# Autodesk Inventor assembly: B_Legs0
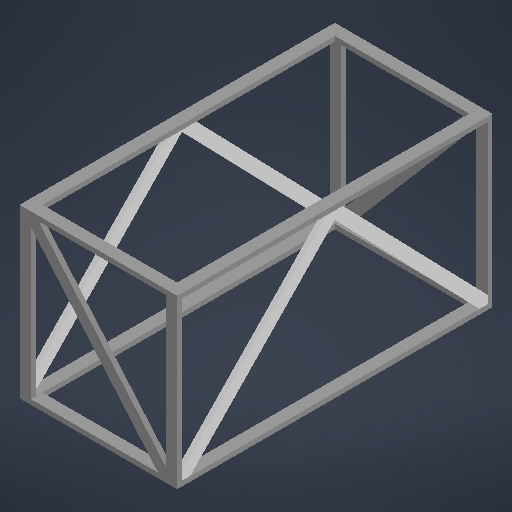
[picture p0: Inventor's stored thumbnail of the model, 512x512]
Saved by Autodesk Inventor 2026 (Build 300175000, 175)
## iProperties
Created: 2024-09-19
Part Number: B_Legs0
Document SubType Name: Assembly
Designer: User
Author: User
## Documents named in this file (7)
- C:\Users\trott\Documents\UofSC-ASME-Tiger-Burn-Design-2025\CAD\Legs\Back Foot\B_Feet.iam
- C:\Users\trott\Documents\UofSC-ASME-Tiger-Burn-Design-2025\CAD\Legs\Back Foot\2x4x120.ipt
- C:\Users\trott\Documents\UofSC-ASME-Tiger-Burn-Design-2025\CAD\Legs\Back Foot\2x4x42.ipt
- C:\Users\trott\Documents\UofSC-ASME-Tiger-Burn-Design-2025\CAD\Legs\Back Foot\2x4x48.ipt
- C:\Users\trott\Documents\UofSC-ASME-Tiger-Burn-Design-2025\CAD\Legs\Back Foot\S_2x4x44.ipt
- C:\Users\trott\Documents\UofSC-ASME-Tiger-Burn-Design-2025\CAD\Legs\Back Foot\S_2x4x65.081.ipt
- C:\Users\trott\Documents\UofSC-ASME-Tiger-Burn-Design-2025\CAD\Legs\Back Foot\S_2x4x68.525.ipt
## Components (18 placed, 6 different names)
1. 2x4x120:1 — Flush:1, Flush:2, Flush:3, Flush:4, Flush:5, Flush:8, Mate:3, Flush:10, Flush:12, Flush:13, Flush:14
2. 2x4x120:2 — Mate:1, Flush:1, Flush:2, Flush:3, Mate:2, Flush:6, Flush:7, Mate:5, Flush:9, Flush:11, Flush:15, Flush:16
3. 2x4x42:1 — Flush:4, Flush:5
4. 2x4x42:2 — Mate:2, Flush:6, Flush:7, Mate:4
5. 2x4x48:1 — Flush:8, Flush:13, Flush:14, Mate:7, Flush:17, Flush:20, Mate:15
6. 2x4x48:2 — Mate:5, Flush:15, Flush:16, Mate:6, Flush:18, Flush:19, Flush:27, Mate:20
7. 2x4x48:3 — Mate:4, Flush:9, Flush:11, Mate:19
8. 2x4x48:4 — Mate:3, Flush:10, Flush:12, Mate:13, Flush:28, Mate:17
9. 2x4x120:3 — Mate:7, Flush:17, Flush:20, Mate:8, Mate:9, Flush:23, Flush:24, Mate:14, Flush:29
10. 2x4x120:4 — Mate:6, Flush:18, Flush:19, Flush:21, Flush:22, Mate:18, Flush:31
11. 2x4x42:3 — Mate:8, Flush:21, Flush:22, Mate:12
12. 2x4x42:4 — Mate:9, Flush:23, Flush:24
13. S_2x4x44:1 — Flush:27
14. S_2x4x44:2 — Mate:12, Mate:13, Flush:28
15. S_2x4x65.081:1 — Mate:16, Flush:30, Mate:17
16. S_2x4x68.525:1 — Mate:14, Flush:29, Mate:15, Mate:16, Flush:30
17. S_2x4x68.525:2 — Mate:18, Flush:31, Mate:19, Mate:21, Flush:32
18. S_2x4x65.081:2 — Mate:20, Mate:21, Flush:32
## Relationships (49: Flush 30, Mate 19)
- Mate:1: 2x4x120:2
- Flush:1: 2x4x120:1 ↔ 2x4x120:2
- Flush:2 (1130.3 mm): 2x4x120:1 ↔ 2x4x120:2
- Flush:3: 2x4x120:1 ↔ 2x4x120:2
- Flush:4: 2x4x120:1 ↔ 2x4x42:1
- Flush:5: 2x4x120:1 ↔ 2x4x42:1
- Mate:2: 2x4x120:2 ↔ 2x4x42:2
- Flush:6: 2x4x120:2 ↔ 2x4x42:2
- Flush:7: 2x4x120:2 ↔ 2x4x42:2
- Flush:8: 2x4x120:1 ↔ 2x4x48:1
- Mate:3: 2x4x120:1 ↔ 2x4x48:4
- Mate:4: 2x4x42:2 ↔ 2x4x48:3
- Mate:5: 2x4x120:2 ↔ 2x4x48:2
- Flush:9: 2x4x120:2 ↔ 2x4x48:3
- Flush:10: 2x4x120:1 ↔ 2x4x48:4
- Flush:11: 2x4x120:2 ↔ 2x4x48:3
- Flush:12: 2x4x120:1 ↔ 2x4x48:4
- Flush:13: 2x4x120:1 ↔ 2x4x48:1
- Flush:14: 2x4x120:1 ↔ 2x4x48:1
- Flush:15: 2x4x120:2 ↔ 2x4x48:2
- Flush:16: 2x4x120:2 ↔ 2x4x48:2
- Mate:6: 2x4x48:2 ↔ 2x4x120:4
- Mate:7: 2x4x48:1 ↔ 2x4x120:3
- Flush:17: 2x4x48:1 ↔ 2x4x120:3
- Flush:18: 2x4x48:2 ↔ 2x4x120:4
- Flush:19: 2x4x48:2 ↔ 2x4x120:4
- Flush:20: 2x4x48:1 ↔ 2x4x120:3
- Mate:8: 2x4x120:3 ↔ 2x4x42:3
- Mate:9: 2x4x120:3 ↔ 2x4x42:4
- Flush:21: 2x4x120:4 ↔ 2x4x42:3
- Flush:22: 2x4x120:4 ↔ 2x4x42:3
- Flush:23: 2x4x120:3 ↔ 2x4x42:4
- Flush:24: 2x4x120:3 ↔ 2x4x42:4
- Flush:27: 2x4x48:2 ↔ S_2x4x44:1
- Mate:12: 2x4x42:3 ↔ S_2x4x44:2
- Mate:13: 2x4x48:4 ↔ S_2x4x44:2
- Flush:28: 2x4x48:4 ↔ S_2x4x44:2
- Mate:14: 2x4x120:3 ↔ S_2x4x68.525:1
- Flush:29: 2x4x120:3 ↔ S_2x4x68.525:1
- Mate:15: 2x4x48:1 ↔ S_2x4x68.525:1
- Mate:16: S_2x4x65.081:1 ↔ S_2x4x68.525:1
- Flush:30: S_2x4x65.081:1 ↔ S_2x4x68.525:1
- Mate:17: 2x4x48:4 ↔ S_2x4x65.081:1
- Mate:18: 2x4x120:4 ↔ S_2x4x68.525:2
- Flush:31: 2x4x120:4 ↔ S_2x4x68.525:2
- Mate:19: 2x4x48:3 ↔ S_2x4x68.525:2
- Mate:20: 2x4x48:2 ↔ S_2x4x65.081:2
- Mate:21: S_2x4x68.525:2 ↔ S_2x4x65.081:2
- Flush:32: S_2x4x68.525:2 ↔ S_2x4x65.081:2
